# Autodesk Inventor assembly: Узел_наклона
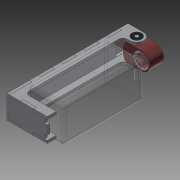
[picture p0: Inventor's stored thumbnail of the model, 180x180]
Saved by Autodesk Inventor 2022 (Build 260153000, 153)
## iProperties
Created: 2025-01-31
Part Number: Узел_наклона
Document SubType Name: Assembly
Designer: Ivan
Author: Ivan
## Documents named in this file (8)
- C:\Users\Ivan\Desktop\Shotter_3\Узел_наклона.iam
- C:\Users\Ivan\Desktop\Shotter_3\Основание.ipt
- C:\Users\Ivan\Desktop\Shotter_3\Вал.ipt
- C:\Users\Ivan\Desktop\Shotter_3\Основание_нижнее.ipt
- C:\Users\Ivan\Desktop\Shotter_3\Подшипник 608 zz.ipt
- C:\Users\Ivan\Desktop\Shotter_3\Стенка_боковая.ipt
- C:\Users\Ivan\Desktop\Shotter_3\Стенка_задняя.ipt
- C:\Users\Ivan\Desktop\Shotter_3\Бутылка_акт.ipt
## Components (9 placed, 7 different names)
1. Вал:1 — Совмещение:5, Совмещение:7, Совмещение:10, Совмещение:11, Совмещение:15
2. Основание_нижнее:1 — Совмещение:13, Заподлицо:3, Заподлицо:4, Заподлицо:7
3. Подшипник 608 zz:1 — Совмещение:7
4. Стенка_боковая:1 — Совмещение:5, Заподлицо:2, Заподлицо:8, Совмещение:20
5. Стенка_задняя:1 — Заподлицо:6, Заподлицо:7, Заподлицо:8
6. Подшипник 608 zz:2 — Совмещение:11, Совмещение:16
7. Стенка_боковая:2 — Совмещение:10, Заподлицо:2, Совмещение:13, Заподлицо:3, Заподлицо:4, Заподлицо:6, Совмещение:17, Угол:1
8. Основание:2 — Совмещение:15, Совмещение:16, Совмещение:17, Совмещение:18, Совмещение:19, Совмещение:20
9. бутылка:1 — Совмещение:18, Совмещение:19, Угол:1
## Relationships (18: Mate 11, Flush 6, Angle 1)
- Совмещение:5 [Mate]: Вал:1 ↔ Стенка_боковая:1
- Совмещение:7 [Mate]: Вал:1 ↔ Подшипник 608 zz:1
- Совмещение:10 [Mate]: Вал:1 ↔ Стенка_боковая:2
- Заподлицо:2 [Flush]: Стенка_боковая:1 ↔ Стенка_боковая:2
- Совмещение:11 [Mate]: Вал:1 ↔ Подшипник 608 zz:2
- Совмещение:13 [Mate]: Основание_нижнее:1 ↔ Стенка_боковая:2
- Заподлицо:3 [Flush]: Основание_нижнее:1 ↔ Стенка_боковая:2
- Заподлицо:4 [Flush]: Основание_нижнее:1 ↔ Стенка_боковая:2
- Заподлицо:6 [Flush]: Стенка_задняя:1 ↔ Стенка_боковая:2
- Заподлицо:7 [Flush]: Основание_нижнее:1 ↔ Стенка_задняя:1
- Совмещение:15 [Mate]: Вал:1 ↔ Основание:2
- Совмещение:16 [Mate]: Подшипник 608 zz:2 ↔ Основание:2
- Совмещение:17 [Mate]: Стенка_боковая:2 ↔ Основание:2
- Совмещение:18 [Mate]: Основание:2 ↔ бутылка:1
- Совмещение:19 [Mate]: Основание:2 ↔ бутылка:1
- Угол:1 [Angle] (0 deg): Стенка_боковая:2 ↔ бутылка:1
- Заподлицо:8 [Flush]: Стенка_боковая:1 ↔ Стенка_задняя:1
- Совмещение:20 [Mate]: Стенка_боковая:1 ↔ Основание:2
